# Autodesk Inventor assembly: Arm 2.0 Assembly
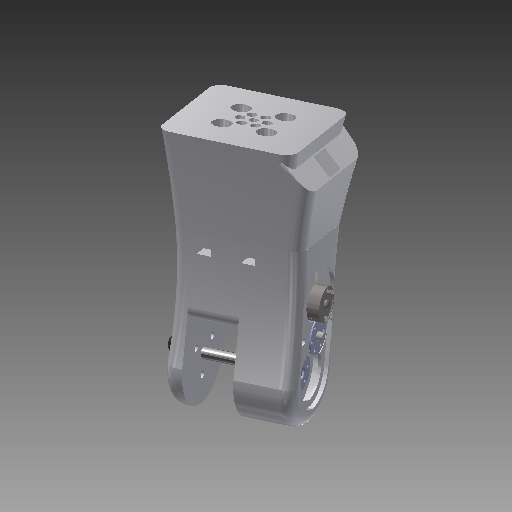
[picture p0: Inventor's stored thumbnail of the model, 512x512]
Saved by Autodesk Inventor 2017 (Build 210142000, 142)
## iProperties
Created: 2017-09-28
Part Number: Arm 2.0 Assembly
Document SubType Name: Assembly
Designer: Zach
Author: Zach
## Documents named in this file (18)
- C:\Users\Dell\Documents\GitHub\tr1\src\Body\Arm Assembly\Wrist Assembly\Wrist Assembly.iam
- C:\Users\Dell\Documents\GitHub\tr1\lib\22x8x8mm Bearing.ipt
- C:\Users\Dell\Documents\GitHub\tr1\lib\12V DC Motor 378-1.ipt
- C:\Users\Dell\Documents\GitHub\tr1\src\Body\Arm Assembly\Wrist Assembly\Steel Rod 8mm x 80mm.ipt
- C:\Users\Dell\Documents\GitHub\tr1\lib\8mm Hub.ipt
- C:\Users\Dell\Documents\GitHub\tr1\lib\4mm mounting hub.ipt
- C:\Users\Dell\Documents\GitHub\tr1\src\Body\Arm Assembly\Wrist Assembly\AA034.ipt
- C:\Users\Dell\Documents\GitHub\tr1\lib\Content Center Files\R2017\en-US\ISO 7045  H\ISO 7045 - M3 x 8 - 4.8 - H - ISO.ipt
- C:\Users\Dell\Documents\GitHub\tr1\src\Body\Arm Assembly\Arm Assembly\Design Accelerator\Spur Gears16.iam
- C:\Users\Dell\Documents\GitHub\tr1\lib\Content Center Files\R2017\en-US\ISO 4018\ISO 4018 - M5 x 10.ipt
- C:\Users\Dell\Documents\GitHub\tr1\lib\Content Center Files\R2017\en-US\ISO 4018\ISO 4018 - M5 x 25.ipt
- C:\Users\Dell\Documents\GitHub\tr1\lib\Content Center Files\R2017\en-US\ISO 7045  H\ISO 7045 - M3 x 12 - 4.8 - H - ISO.ipt
- C:\Users\Dell\Documents\GitHub\tr1\src\Body\Arm Assembly\Wrist Assembly\AA049.ipt
- C:\Users\Dell\Documents\GitHub\tr1\lib\Content Center Files\R2017\en-US\ISO 4035(2)\ISO 4035 - M5 - ISO.ipt
- C:\Users\Dell\Documents\GitHub\tr1\lib\6mm Mounting Hub.ipt
- C:\Users\Dell\Documents\GitHub\tr1\lib\EMS22XXX-D28-LSX.ipt
- C:\Users\Dell\Documents\GitHub\tr1\src\Body\Arm Assembly\Wrist Assembly\AA045b.ipt
- C:\Users\Dell\Documents\GitHub\tr1\src\Body\Arm Assembly\Wrist Assembly\AASG09a.ipt
## Components (37 placed, 17 different names)
1. AA034:1 — Mate:534, Mate:535, Mate:879, Mate:880, Mate:881, Mate:882, Mate:883, Mate:884, Mate:885, Mate:886, Mate:964, Mate:965, Mate:966, Mate:967, Mate:968, Mate:969, Mate:970, Mate:971, Mate:972, Mate:973, Mate:974, Mate:975, Mate:1213, Mate:1256, Mate:1310, Mate:1311
2. AA045b:1 — Mate:1211, Mate:1212, Angle:27, Mate:1213, Mate:1214, Mate:1215, Mate:1216, Mate:1218, Mate:1219, Flush:37, Mate:1221, Mate:1224, Mate:1225, Mate:1235, Mate:1264, Mate:1265, Mate:1310, Mate:1311, Mate:1327
3. AA049:1 — Mate:783, Mate:786, Mate:787, Mate:788, Mate:789, Mate:790, Mate:791, Mate:1218
4. 22x8x8mm Bearing:5 — Mate:186, Mate:1265
5. 22x8x8mm Bearing:6 — Mate:187, Mate:1264
6. Steel Rod 8mm x 80mm:1 — Mate:186, Mate:187, Mate:721, Mate:724, Mate:783, Mate:1216, Flush:37, Mate:1234
7. 12V DC Motor 378-1:3 — Mate:714, Mate:778, Mate:779, Mate:1224, Mate:1225, Mate:1326
8. 6mm Mounting Hub:10 — Mate:1228, Mate:1323
9. 8mm Hub:2 — Mate:534, Mate:535
10. 8mm Hub:8 — Mate:721, Mate:1234, Mate:1324, Mate:1325
11. 4mm mounting hub:8 — Mate:714, Mate:1330
12. EMS22XXX-D28-LSX:6 — Mate:1211, Mate:1212, Angle:27, Mate:1228, Mate:1267
13. AASG10 [sub-assembly] — Mate:724, Mate:1221, Mate:1235, Mate:1267, Mate:1323, Mate:1324, Mate:1325
14. ISO 7045 H M3 x 8 - 4.8 - H:5 — Mate:778
15. ISO 7045 H M3 x 8 - 4.8 - H:6 — Mate:779
16. ISO 7045 H M3 x 8 - 4.8 - H:27 — Mate:965, Mate:972
17. ISO 7045 H M3 x 8 - 4.8 - H:28 — Mate:964, Mate:973
18. ISO 7045 H M3 x 8 - 4.8 - H:29 — Mate:966, Mate:971
19. ISO 7045 H M3 x 8 - 4.8 - H:30 — Mate:967, Mate:970, Mate:1256
20. ISO 7045 H M3 x 8 - 4.8 - H:31 — Mate:969, Mate:975
21. ISO 7045 H M3 x 8 - 4.8 - H:32 — Mate:968, Mate:974
22. ISO 7045 H M3 x 12 - 4.8 - H:4 — Mate:1331, Mate:1332
23. ISO 7045 H M3 x 12 - 4.8 - H:5 — Mate:1328, Mate:1329
24. ISO 7045 H M3 x 12 - 4.8 - H:6 — Mate:1335, Mate:1336
25. ISO 7045 H M3 x 12 - 4.8 - H:7 — Mate:1333, Mate:1334
26. ISO 4035 M5:5 — Mate:985
27. ISO 4035 M5:6 — Mate:984
28. ISO 4035 M5:7 — Mate:989
29. ISO 4035 M5:8 — Mate:988
30. ISO 4018 M5 x 10:3 — Mate:787, Mate:790
31. ISO 4018 M5 x 10:4 — Mate:788, Mate:791
32. ISO 4018 M5 x 10:5 — Mate:786, Mate:789, Mate:1219
33. ISO 4018 M5 x 25:40 — Mate:882, Mate:883, Mate:984
34. ISO 4018 M5 x 25:41 — Mate:880, Mate:886, Mate:988, Mate:1214
35. ISO 4018 M5 x 25:42 — Mate:879, Mate:885, Mate:985
36. ISO 4018 M5 x 25:43 — Mate:881, Mate:884, Mate:989, Mate:1215
37. Spur Gear2:1 — Mate:1326, Mate:1327, Mate:1328, Mate:1329, Mate:1330, Mate:1331, Mate:1332, Mate:1333, Mate:1334, Mate:1335, Mate:1336
## Relationships (76: Mate 74, Angle 1, Flush 1)
- Mate:186: 22x8x8mm Bearing:5 ↔ Steel Rod 8mm x 80mm:1
- Mate:187: 22x8x8mm Bearing:6 ↔ Steel Rod 8mm x 80mm:1
- Mate:534: AA034:1 ↔ 8mm Hub:2
- Mate:535: AA034:1 ↔ 8mm Hub:2
- Mate:714: 12V DC Motor 378-1:3 ↔ 4mm mounting hub:8
- Mate:721: Steel Rod 8mm x 80mm:1 ↔ 8mm Hub:8
- Mate:724: Steel Rod 8mm x 80mm:1 ↔ AASG10
- Mate:778: 12V DC Motor 378-1:3 ↔ ISO 7045 H M3 x 8 - 4.8 - H:5
- Mate:779: 12V DC Motor 378-1:3 ↔ ISO 7045 H M3 x 8 - 4.8 - H:6
- Mate:783: AA049:1 ↔ Steel Rod 8mm x 80mm:1
- Mate:786: AA049:1 ↔ ISO 4018 M5 x 10:5
- Mate:787: AA049:1 ↔ ISO 4018 M5 x 10:3
- Mate:788: AA049:1 ↔ ISO 4018 M5 x 10:4
- Mate:789: AA049:1 ↔ ISO 4018 M5 x 10:5
- Mate:790: AA049:1 ↔ ISO 4018 M5 x 10:3
- Mate:791: AA049:1 ↔ ISO 4018 M5 x 10:4
- Mate:879: AA034:1 ↔ ISO 4018 M5 x 25:42
- Mate:880: AA034:1 ↔ ISO 4018 M5 x 25:41
- Mate:881: AA034:1 ↔ ISO 4018 M5 x 25:43
- Mate:882: AA034:1 ↔ ISO 4018 M5 x 25:40
- Mate:883: AA034:1 ↔ ISO 4018 M5 x 25:40
- Mate:884: AA034:1 ↔ ISO 4018 M5 x 25:43
- Mate:885: AA034:1 ↔ ISO 4018 M5 x 25:42
- Mate:886: AA034:1 ↔ ISO 4018 M5 x 25:41
- Mate:964: AA034:1 ↔ ISO 7045 H M3 x 8 - 4.8 - H:28
- Mate:965: AA034:1 ↔ ISO 7045 H M3 x 8 - 4.8 - H:27
- Mate:966: AA034:1 ↔ ISO 7045 H M3 x 8 - 4.8 - H:29
- Mate:967: AA034:1 ↔ ISO 7045 H M3 x 8 - 4.8 - H:30
- Mate:968: AA034:1 ↔ ISO 7045 H M3 x 8 - 4.8 - H:32
- Mate:969: AA034:1 ↔ ISO 7045 H M3 x 8 - 4.8 - H:31
- Mate:970: AA034:1 ↔ ISO 7045 H M3 x 8 - 4.8 - H:30
- Mate:971: AA034:1 ↔ ISO 7045 H M3 x 8 - 4.8 - H:29
- Mate:972: AA034:1 ↔ ISO 7045 H M3 x 8 - 4.8 - H:27
- Mate:973: AA034:1 ↔ ISO 7045 H M3 x 8 - 4.8 - H:28
- Mate:974: AA034:1 ↔ ISO 7045 H M3 x 8 - 4.8 - H:32
- Mate:975: AA034:1 ↔ ISO 7045 H M3 x 8 - 4.8 - H:31
- Mate:984: ISO 4035 M5:6 ↔ ISO 4018 M5 x 25:40
- Mate:985: ISO 4035 M5:5 ↔ ISO 4018 M5 x 25:42
- Mate:988: ISO 4035 M5:8 ↔ ISO 4018 M5 x 25:41
- Mate:989: ISO 4035 M5:7 ↔ ISO 4018 M5 x 25:43
- Mate:1211: AA045b:1 ↔ EMS22XXX-D28-LSX:6
- Mate:1212: AA045b:1 ↔ EMS22XXX-D28-LSX:6
- Angle:27 (0 deg): AA045b:1 ↔ EMS22XXX-D28-LSX:6
- Mate:1213: AA034:1 ↔ AA045b:1
- Mate:1214: AA045b:1 ↔ ISO 4018 M5 x 25:41
- Mate:1215: AA045b:1 ↔ ISO 4018 M5 x 25:43
- Mate:1216: AA045b:1 ↔ Steel Rod 8mm x 80mm:1
- Mate:1218: AA045b:1 ↔ AA049:1
- Mate:1219: AA045b:1 ↔ ISO 4018 M5 x 10:5
- Flush:37 (-2.5 mm): AA045b:1 ↔ Steel Rod 8mm x 80mm:1
- Mate:1221: AA045b:1 ↔ AASG10
- Mate:1224: AA045b:1 ↔ 12V DC Motor 378-1:3
- Mate:1225: AA045b:1 ↔ 12V DC Motor 378-1:3
- Mate:1228: 6mm Mounting Hub:10 ↔ EMS22XXX-D28-LSX:6
- Mate:1234: Steel Rod 8mm x 80mm:1 ↔ 8mm Hub:8
- Mate:1235: AA045b:1 ↔ AASG10
- Mate:1256: AA034:1 ↔ ISO 7045 H M3 x 8 - 4.8 - H:30
- Mate:1264: AA045b:1 ↔ 22x8x8mm Bearing:6
- Mate:1265: AA045b:1 ↔ 22x8x8mm Bearing:5
- Mate:1267: EMS22XXX-D28-LSX:6 ↔ AASG10
- Mate:1310: AA034:1 ↔ AA045b:1
- Mate:1311: AA034:1 ↔ AA045b:1
- Mate:1323: 6mm Mounting Hub:10 ↔ AASG10
- Mate:1324: 8mm Hub:8 ↔ AASG10
- Mate:1325: 8mm Hub:8 ↔ AASG10
- Mate:1326: 12V DC Motor 378-1:3 ↔ Spur Gear2:1
- Mate:1327: AA045b:1 ↔ Spur Gear2:1
- Mate:1328: ISO 7045 H M3 x 12 - 4.8 - H:5 ↔ Spur Gear2:1
- Mate:1329: ISO 7045 H M3 x 12 - 4.8 - H:5 ↔ Spur Gear2:1
- Mate:1330: 4mm mounting hub:8 ↔ Spur Gear2:1
- Mate:1331: ISO 7045 H M3 x 12 - 4.8 - H:4 ↔ Spur Gear2:1
- Mate:1332: ISO 7045 H M3 x 12 - 4.8 - H:4 ↔ Spur Gear2:1
- Mate:1333: ISO 7045 H M3 x 12 - 4.8 - H:7 ↔ Spur Gear2:1
- Mate:1334: ISO 7045 H M3 x 12 - 4.8 - H:7 ↔ Spur Gear2:1
- Mate:1335: ISO 7045 H M3 x 12 - 4.8 - H:6 ↔ Spur Gear2:1
- Mate:1336: ISO 7045 H M3 x 12 - 4.8 - H:6 ↔ Spur Gear2:1
